# Autodesk Inventor assembly: A006
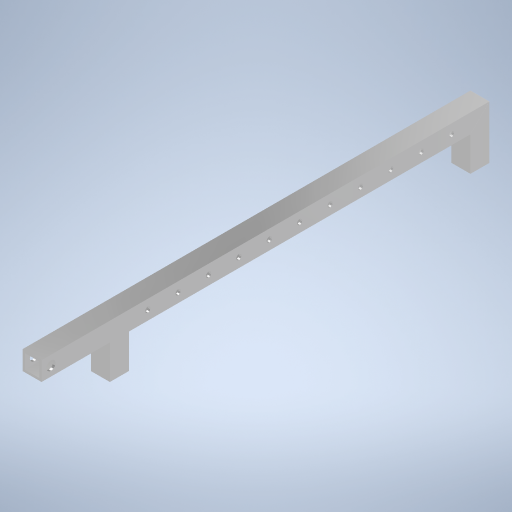
[picture p0: Inventor's stored thumbnail of the model, 512x512]
Saved by Autodesk Inventor 2023 (Build 270158000, 158)
## iProperties
Created: 2022-08-23
Part Number: A006
Document SubType Name: Assembly
Designer: D.C. Eksteen
Mass: 317.072 g
Surface Area: 1206.83 cm^2
Volume: 117.434 cm^3
Density: 2.7 g/cm^3
Author: D.C. Eksteen
Title: RIGHT FRONT FRAME ASSEMBLY
## Documents named in this file (4)
- C:\Users\dylan\Desktop\Skripsie-2022\Design\CAD\FRONT FRAME RIGHT.iam
- C:\Users\dylan\Desktop\Skripsie-2022\Design\CAD\FRONT FRAME PLAIN RISER.ipt
- C:\Users\dylan\Desktop\Skripsie-2022\Design\CAD\FRONT FRAME RISER.ipt
- C:\Users\dylan\Desktop\Skripsie-2022\Design\CAD\FRONT FRAME RIGHT BRACKET.ipt
## Components (3 placed, 3 different names)
1. FRONT FRAME PLAIN RISER:1
2. FRONT FRAME RISER:1
3. FRONT FRAME RIGHT BRACKET:1
## Relationships (7: Mate 5, Flush 2)
- [Mate] (450 mm): FRONT FRAME PLAIN RISER:1 ↔ FRONT FRAME RISER:1
- [Mate]: FRONT FRAME RISER:1 ↔ FRONT FRAME RIGHT BRACKET:1
- [Flush]: FRONT FRAME RISER:1 ↔ FRONT FRAME RIGHT BRACKET:1
- [Mate]: FRONT FRAME PLAIN RISER:1 ↔ FRONT FRAME RIGHT BRACKET:1
- [Flush]: FRONT FRAME PLAIN RISER:1 ↔ FRONT FRAME RIGHT BRACKET:1
- [Mate]: FRONT FRAME PLAIN RISER:1
- [Mate]: FRONT FRAME RIGHT BRACKET:1
